# Autodesk Inventor assembly: v2RevA
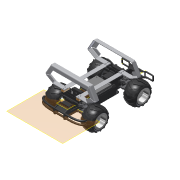
[picture p0: Inventor's stored thumbnail of the model, 180x180]
Saved by Autodesk Inventor 2015 (Build 190159000, 159)
## iProperties
Created: 2013-12-30
Part Number: v2RevA
Document SubType Name: Assembly
Designer: davidgitz
Author: davidgitz
## Documents named in this file (6)
- C:\SharedDrive\Dropbox\ICARUS\Rover\MECHANICAL\810002_ASY-FAST ROVER v2\813004_FAST ROVER v2 CHASSIS\813004_FAST ROVER v2 CHASSIS.iam
- C:\SharedDrive\Dropbox\ICARUS\Rover\MECHANICAL\810002_ASY-FAST ROVER v2\813004_FAST ROVER v2 CHASSIS\813005_Hummer H2 Chassis\813005_Hummer H2 Chassis.iam
- C:\SharedDrive\Dropbox\ICARUS\Rover\MECHANICAL\810002_ASY-FAST ROVER v2\813004_FAST ROVER v2 CHASSIS\800000_Frame Block.ipt
- C:\SharedDrive\Dropbox\ICARUS\Rover\MECHANICAL\810002_ASY-FAST ROVER v2\813004_FAST ROVER v2 CHASSIS\571001_Frame Member.ipt
- C:\SharedDrive\Dropbox\ICARUS\Rover\MECHANICAL\810002_ASY-FAST ROVER v2\813004_FAST ROVER v2 CHASSIS\571002_Cage Frame.ipt
- C:\SharedDrive\Dropbox\ICARUS\Rover\MECHANICAL\810002_ASY-FAST ROVER v2\813004_FAST ROVER v2 CHASSIS\813005_Hummer H2 Chassis\FrontBumper.ipt
## Components (8 placed, 5 different names)
1. 813005_Hummer H2 Chassis:1 [sub-assembly] — Flush:1, Flush:2, Flush:3, Mate:1, Mate:3, Angle:1, Mate:4, Mate:8, Flush:15, Mate:11, Flush:16
2. 571001_Frame Member:1 — Mate:1, Flush:4, Flush:5, Mate:2, Flush:8, Insert:1, Flush:10
3. 800000_Frame Block:1 — Flush:4, Flush:5, Mate:2, Mate:3, Angle:1, Flush:9
4. 571001_Frame Member:2 — Mate:4, Flush:6, Mate:5, Flush:7, Flush:8, Insert:2
5. 800000_Frame Block:2 — Flush:6, Mate:5, Flush:7, Flush:9, Flush:11
6. 571002_Cage Frame:1 — Insert:1, Flush:11
7. 571002_Cage Frame:2 — Insert:2, Flush:10
8. FrontBumper:1 — Flush:15, Mate:11, Flush:16
## Relationships (23: Flush 13, Mate 7, Insert 2, Angle 1)
- Flush:1: 813005_Hummer H2 Chassis:1
- Flush:2: 813005_Hummer H2 Chassis:1
- Flush:3: 813005_Hummer H2 Chassis:1
- Mate:1: 813005_Hummer H2 Chassis:1 ↔ 571001_Frame Member:1
- Flush:4: 571001_Frame Member:1 ↔ 800000_Frame Block:1
- Flush:5: 571001_Frame Member:1 ↔ 800000_Frame Block:1
- Mate:2: 571001_Frame Member:1 ↔ 800000_Frame Block:1
- Mate:3: 813005_Hummer H2 Chassis:1 ↔ 800000_Frame Block:1
- Angle:1 (0 deg): 813005_Hummer H2 Chassis:1 ↔ 800000_Frame Block:1
- Mate:4: 813005_Hummer H2 Chassis:1 ↔ 571001_Frame Member:2
- Flush:6: 571001_Frame Member:2 ↔ 800000_Frame Block:2
- Mate:5: 571001_Frame Member:2 ↔ 800000_Frame Block:2
- Flush:7: 571001_Frame Member:2 ↔ 800000_Frame Block:2
- Flush:8: 571001_Frame Member:1 ↔ 571001_Frame Member:2
- Flush:9: 800000_Frame Block:1 ↔ 800000_Frame Block:2
- Insert:1: 571001_Frame Member:1 ↔ 571002_Cage Frame:1
- Insert:2: 571001_Frame Member:2 ↔ 571002_Cage Frame:2
- Flush:10: 571001_Frame Member:1 ↔ 571002_Cage Frame:2
- Flush:11: 800000_Frame Block:2 ↔ 571002_Cage Frame:1
- Mate:8: 813005_Hummer H2 Chassis:1
- Flush:15: 813005_Hummer H2 Chassis:1 ↔ FrontBumper:1
- Mate:11: 813005_Hummer H2 Chassis:1 ↔ FrontBumper:1
- Flush:16: 813005_Hummer H2 Chassis:1 ↔ FrontBumper:1
